# Autodesk Inventor assembly: test-model-28BYJ_2
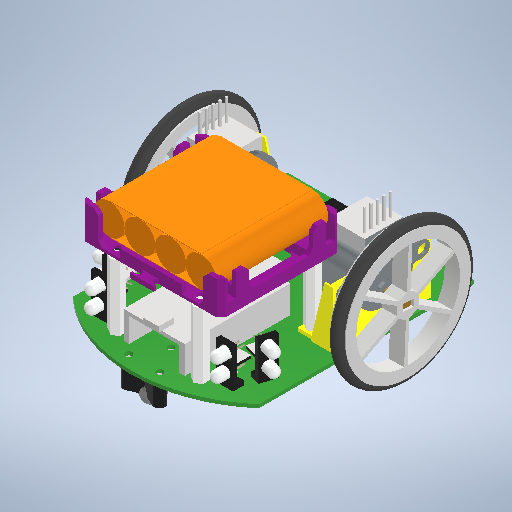
[picture p0: Inventor's stored thumbnail of the model, 512x512]
Saved by Autodesk Inventor 2025.3 (Build 293356000, 356)
## iProperties
Created: 2025-05-29
Part Number: test-model-28BYJ_2
Document SubType Name: Assembly
Designer: yamashita1
Author: yamashita1
## Documents named in this file (14)
- G:\マイドライブ\project\micro-mouse\3D-Model\test-model-28BYJ_2.iam
- G:\マイドライブ\project\micro-mouse\3D-Model\BallCaster-H16.ipt
- G:\マイドライブ\project\micro-mouse\3D-Model\Photo-Sensor.iam
- G:\マイドライブ\project\micro-mouse\3D-Model\ESP32-DevKitC.ipt
- G:\マイドライブ\project\micro-mouse\3D-Model\AQM1602Y.ipt
- G:\マイドライブ\project\micro-mouse\3D-Model\BaseBoard-stp3.ipt
- G:\マイドライブ\project\micro-mouse\3D-Model\Spacer-M3H30.ipt
- G:\マイドライブ\project\micro-mouse\3D-Model\28BYJ-48_Braket3.ipt
- G:\マイドライブ\project\micro-mouse\3D-Model\28BYJ-48.ipt
- G:\マイドライブ\project\micro-mouse\3D-Model\Wheel-D63C.ipt
- G:\マイドライブ\project\micro-mouse\3D-Model\O-ring_D63.ipt
- G:\マイドライブ\project\micro-mouse\3D-Model\Ground.ipt
- G:\マイドライブ\project\micro-mouse\3D-Model\Battery-Holder3-1x4.ipt
- G:\マイドライブ\project\micro-mouse\3D-Model\NiMH-Battery.ipt
## Components (23 placed, 13 different names)
1. BallCaster-H16:1 — メイト:7, メイト:8, メイト:9
2. Photo-Sensor:1 [sub-assembly] — メイト:15
3. Photo-Sensor:2 [sub-assembly] — メイト:14
4. Photo-Sensor:3 [sub-assembly] — メイト:12
5. Photo-Sensor:4 [sub-assembly] — メイト:13
6. ESP32-DevKitC:1 — メイト:10
7. AQM1602Y:1 — メイト:11
8. BaseBoard-stp3:1 — メイト:7, メイト:8, メイト:9, メイト:10, メイト:11, メイト:12, メイト:13, メイト:14, メイト:15, メイト:26, メイト:27, メイト:28, メイト:29, メイト:30, メイト:31, メイト:32, メイト:33, メイト:34, メイト:35
9. Spacer-M3H30:1 — メイト:26, メイト:28
10. Spacer-M3H30:2 — メイト:27, メイト:29, メイト:55
11. Spacer-M3H30:3 — メイト:50, メイト:51, メイト:54, メイト:56
12. Spacer-M3H30:4 — メイト:52, メイト:53
13. 28BYJ-48_Braket3:1 — メイト:30, メイト:31, メイト:32, メイト:36, メイト:37, メイト:38, メイト:50, メイト:51
14. 28BYJ-48_Braket3:2 — メイト:33, メイト:34, メイト:35, メイト:39, メイト:40, メイト:41, メイト:52, メイト:53
15. 28BYJ-48:1 — メイト:36, メイト:37, メイト:38, メイト:42, メイト:43
16. 28BYJ-48:2 — メイト:39, メイト:40, メイト:41, メイト:44, メイト:45
17. Wheel-D63C:1 — メイト:42, メイト:43, メイト:46, メイト:47
18. Wheel-D63C:2 — メイト:44, メイト:45, メイト:48, メイト:49
19. O-ring_D63:1 — メイト:46, メイト:47
20. O-ring_D63:2 — メイト:48, メイト:49
21. Ground:1
22. Battery-Holder3-1x4:1 — メイト:54, メイト:55, メイト:56, メイト:57, メイト:58
23. NiMH-Battery:1 — メイト:57, メイト:58
## Relationships (42: Mate 42)
- メイト:7 [Mate]: BallCaster-H16:1 ↔ BaseBoard-stp3:1
- メイト:8 [Mate]: BallCaster-H16:1 ↔ BaseBoard-stp3:1
- メイト:9 [Mate]: BallCaster-H16:1 ↔ BaseBoard-stp3:1
- メイト:10 [Mate]: ESP32-DevKitC:1 ↔ BaseBoard-stp3:1
- メイト:11 [Mate]: AQM1602Y:1 ↔ BaseBoard-stp3:1
- メイト:12 [Mate]: Photo-Sensor:3 ↔ BaseBoard-stp3:1
- メイト:13 [Mate]: Photo-Sensor:4 ↔ BaseBoard-stp3:1
- メイト:14 [Mate]: Photo-Sensor:2 ↔ BaseBoard-stp3:1
- メイト:15 [Mate]: Photo-Sensor:1 ↔ BaseBoard-stp3:1
- メイト:26 [Mate]: BaseBoard-stp3:1 ↔ Spacer-M3H30:1
- メイト:27 [Mate]: BaseBoard-stp3:1 ↔ Spacer-M3H30:2
- メイト:28 [Mate]: BaseBoard-stp3:1 ↔ Spacer-M3H30:1
- メイト:29 [Mate]: BaseBoard-stp3:1 ↔ Spacer-M3H30:2
- メイト:30 [Mate]: BaseBoard-stp3:1 ↔ 28BYJ-48_Braket3:1
- メイト:31 [Mate]: BaseBoard-stp3:1 ↔ 28BYJ-48_Braket3:1
- メイト:32 [Mate]: BaseBoard-stp3:1 ↔ 28BYJ-48_Braket3:1
- メイト:33 [Mate]: BaseBoard-stp3:1 ↔ 28BYJ-48_Braket3:2
- メイト:34 [Mate]: BaseBoard-stp3:1 ↔ 28BYJ-48_Braket3:2
- メイト:35 [Mate]: BaseBoard-stp3:1 ↔ 28BYJ-48_Braket3:2
- メイト:36 [Mate]: 28BYJ-48_Braket3:1 ↔ 28BYJ-48:1
- メイト:37 [Mate]: 28BYJ-48_Braket3:1 ↔ 28BYJ-48:1
- メイト:38 [Mate]: 28BYJ-48_Braket3:1 ↔ 28BYJ-48:1
- メイト:39 [Mate]: 28BYJ-48_Braket3:2 ↔ 28BYJ-48:2
- メイト:40 [Mate]: 28BYJ-48_Braket3:2 ↔ 28BYJ-48:2
- メイト:41 [Mate]: 28BYJ-48_Braket3:2 ↔ 28BYJ-48:2
- メイト:42 [Mate]: 28BYJ-48:1 ↔ Wheel-D63C:1
- メイト:43 [Mate]: 28BYJ-48:1 ↔ Wheel-D63C:1
- メイト:44 [Mate]: 28BYJ-48:2 ↔ Wheel-D63C:2
- メイト:45 [Mate]: 28BYJ-48:2 ↔ Wheel-D63C:2
- メイト:46 [Mate]: Wheel-D63C:1 ↔ O-ring_D63:1
- メイト:47 [Mate]: Wheel-D63C:1 ↔ O-ring_D63:1
- メイト:48 [Mate]: Wheel-D63C:2 ↔ O-ring_D63:2
- メイト:49 [Mate]: Wheel-D63C:2 ↔ O-ring_D63:2
- メイト:50 [Mate]: Spacer-M3H30:3 ↔ 28BYJ-48_Braket3:1
- メイト:51 [Mate]: Spacer-M3H30:3 ↔ 28BYJ-48_Braket3:1
- メイト:52 [Mate]: Spacer-M3H30:4 ↔ 28BYJ-48_Braket3:2
- メイト:53 [Mate]: Spacer-M3H30:4 ↔ 28BYJ-48_Braket3:2
- メイト:54 [Mate]: Spacer-M3H30:3 ↔ Battery-Holder3-1x4:1
- メイト:55 [Mate]: Spacer-M3H30:2 ↔ Battery-Holder3-1x4:1
- メイト:56 [Mate]: Spacer-M3H30:3 ↔ Battery-Holder3-1x4:1
- メイト:57 [Mate]: Battery-Holder3-1x4:1 ↔ NiMH-Battery:1
- メイト:58 [Mate]: Battery-Holder3-1x4:1 ↔ NiMH-Battery:1
